# Autodesk Inventor assembly: Drone
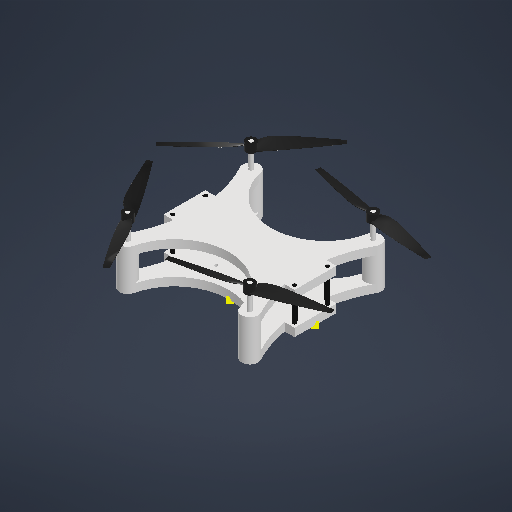
[picture p0: Inventor's stored thumbnail of the model, 512x512]
Saved by Autodesk Inventor 2026.1 (Build 301233000, 233)
## iProperties
Created: 2025-11-21
Part Number: Drone
Document SubType Name: Assembly
Designer: auric
Author: auric
## Documents named in this file (4)
- C:\Users\auric\Downloads\Drone.iam
- C:\Users\auric\Downloads\drone base.ipt
- C:\Users\auric\Downloads\PROPELLER.ipt
- C:\Users\auric\Downloads\DRONE SCREW.ipt
## Components (9 placed, 3 different names)
1. drone base:1 — Rotational:1, Rotational:2, Rotational:3, Rotational:4, Mate:1, Flush:1, Mate:2, Flush:2, Mate:3, Flush:3, Mate:4, Flush:4
2. PROPELLER:1 — Rotational:1
3. PROPELLER:2 — Rotational:2
4. PROPELLER:3 — Rotational:4
5. PROPELLER:4 — Rotational:3
6. DRONE SCREW:1 — Mate:1, Flush:1
7. DRONE SCREW:2 — Mate:3, Flush:3
8. DRONE SCREW:3 — Mate:4, Flush:4
9. DRONE SCREW:4 — Mate:2, Flush:2
## Relationships (12: RevoluteJoint 4, Mate 4, Flush 4)
- Rotational:1 [RevoluteJoint]: drone base:1 ↔ PROPELLER:1
- Rotational:2 [RevoluteJoint]: drone base:1 ↔ PROPELLER:2
- Rotational:3 [RevoluteJoint]: drone base:1 ↔ PROPELLER:4
- Rotational:4 [RevoluteJoint]: drone base:1 ↔ PROPELLER:3
- Mate:1: drone base:1 ↔ DRONE SCREW:1
- Flush:1: drone base:1 ↔ DRONE SCREW:1
- Mate:2: drone base:1 ↔ DRONE SCREW:4
- Flush:2: drone base:1 ↔ DRONE SCREW:4
- Mate:3: drone base:1 ↔ DRONE SCREW:2
- Flush:3: drone base:1 ↔ DRONE SCREW:2
- Mate:4: drone base:1 ↔ DRONE SCREW:3
- Flush:4: drone base:1 ↔ DRONE SCREW:3
